# Autodesk Inventor assembly: Throttle Assembly
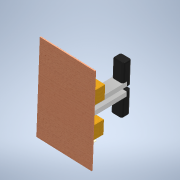
[picture p0: Inventor's stored thumbnail of the model, 180x180]
Saved by Autodesk Inventor 2020.4 (Build 244396000, 396)
## iProperties
Created: 2022-04-16
Part Number: Throttle Assembly
Document SubType Name: Assembly
Designer: Gurkin
Author: Gurkin
## Documents named in this file (6)
- Z:\Class\Skripsie\CAD\Throttle Assembly.iam
- Z:\Class\Skripsie\CAD\Throttle Arm.ipt
- Z:\Class\Skripsie\CAD\Throttle Handler.ipt
- Z:\Class\Skripsie\CAD\Pin Block.ipt
- Z:\Class\Skripsie\CAD\Base.ipt
- Z:\Class\Skripsie\CAD\POT mount.ipt
## Components (9 placed, 5 different names)
1. Base:1 — Flush:2, Mate:7, Mate:12, Flush:5, Mate:16, Mate:19, Flush:6
2. Pin Block:1 — Mate:4, Mate:6, Mate:7, Flush:4, Flush:5, Mate:17, Mate:18
3. Throttle Arm:1 — Mate:1, Mate:2, Mate:4, Mate:6, Flush:1, Mate:13
4. Throttle Handler:1 — Mate:1, Mate:2, Flush:1
5. Throttle Arm:2 — Mate:13
6. Throttle Handler:2
7. Pin Block:2 — Mate:12, Flush:4, Mate:14, Mate:15
8. POT mount:1 — Mate:14, Mate:15, Mate:16
9. POT mount:2 — Mate:17, Mate:18, Mate:19, Flush:6
## Relationships (23: Mate 17, Flush 6)
- Mate:1: Throttle Arm:1 ↔ Throttle Handler:1
- Mate:2: Throttle Arm:1 ↔ Throttle Handler:1
- Mate:4 (10 mm): Pin Block:1 ↔ Throttle Arm:1
- Mate:6: Pin Block:1 ↔ Throttle Arm:1
- Flush:1: Throttle Arm:1 ↔ Throttle Handler:1
- Flush:2: Base:1
- Mate:7: Base:1 ↔ Pin Block:1
- [Mate]: Throttle Arm:2 ↔ Throttle Handler:2
- [Mate]: Throttle Arm:2 ↔ Throttle Handler:2
- [Mate] (10 mm): Throttle Arm:2 ↔ Pin Block:2
- [Mate]: Throttle Arm:2 ↔ Pin Block:2
- [Flush]: Throttle Arm:2 ↔ Throttle Handler:2
- Mate:12: Base:1 ↔ Pin Block:2
- Flush:4: Pin Block:1 ↔ Pin Block:2
- Flush:5 (20 mm): Base:1 ↔ Pin Block:1
- Mate:13 (20 mm): Throttle Arm:1 ↔ Throttle Arm:2
- Mate:14: Pin Block:2 ↔ POT mount:1
- Mate:15 (25 mm): Pin Block:2 ↔ POT mount:1
- Mate:16: Base:1 ↔ POT mount:1
- Mate:17: Pin Block:1 ↔ POT mount:2
- Mate:18 (25 mm): Pin Block:1 ↔ POT mount:2
- Mate:19: Base:1 ↔ POT mount:2
- Flush:6 (30 mm): Base:1 ↔ POT mount:2
## Named parameters: d10_d6 = 0 mm, d11_d7 = 0 mm, d12_d0 = 0 mm, d13_d2 = 0 mm, d14_d4 = 10 mm
